# Autodesk Inventor assembly: short wall
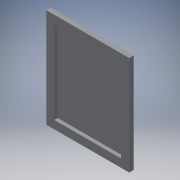
[picture p0: Inventor's stored thumbnail of the model, 180x180]
Saved by Autodesk Inventor 2017 (Build 210142000, 142)
## iProperties
Created: 2019-05-06
Part Number: short wall
Document SubType Name: Assembly
Designer: Roman
Author: Roman
## Documents named in this file (4)
- C:\Users\Roman\Documents\CAD\tegu rev2\upper walls\short wall\short wall.iam
- C:\Users\Roman\Documents\CAD\tegu rev2\upper walls\short wall\upper short wall h bar.ipt
- C:\Users\Roman\Documents\CAD\tegu rev2\upper walls\short wall\upper short wall v bar.ipt
- C:\Users\Roman\Documents\CAD\tegu rev2\upper walls\short wall\upper short wall back.ipt
## Components (5 placed, 3 different names)
1. upper short wall h bar:1 — Mate:1, Flush:1, Flush:2, Mate:2, Flush:3, Flush:4, Mate:4, Flush:7, Flush:8
2. upper short wall h bar:2 — Mate:3, Flush:5, Flush:6
3. upper short wall v bar:1 — Mate:1, Flush:1, Flush:2
4. upper short wall v bar:2 — Mate:2, Flush:3, Flush:4, Mate:3, Flush:5, Flush:6
5. upper short wall back:1 — Mate:4, Flush:7, Flush:8
## Relationships (12: Flush 8, Mate 4)
- Mate:1: upper short wall h bar:1 ↔ upper short wall v bar:1
- Flush:1: upper short wall h bar:1 ↔ upper short wall v bar:1
- Flush:2: upper short wall h bar:1 ↔ upper short wall v bar:1
- Mate:2: upper short wall h bar:1 ↔ upper short wall v bar:2
- Flush:3: upper short wall h bar:1 ↔ upper short wall v bar:2
- Flush:4: upper short wall h bar:1 ↔ upper short wall v bar:2
- Mate:3: upper short wall h bar:2 ↔ upper short wall v bar:2
- Flush:5: upper short wall h bar:2 ↔ upper short wall v bar:2
- Flush:6: upper short wall h bar:2 ↔ upper short wall v bar:2
- Mate:4: upper short wall h bar:1 ↔ upper short wall back:1
- Flush:7: upper short wall h bar:1 ↔ upper short wall back:1
- Flush:8: upper short wall h bar:1 ↔ upper short wall back:1
